# Autodesk Inventor assembly: RoboCinWheel
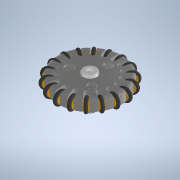
[picture p0: Inventor's stored thumbnail of the model, 180x180]
Saved by Autodesk Inventor 2020.4 (Build 244396000, 396)
## iProperties
Created: 2021-05-01
Part Number: RoboCinWheel
Document SubType Name: Assembly
Designer: Acer
Author: Acer
## Documents named in this file (10)
- C:\Users\Acer\Documents\MATLAB\Doutorado\CAD\Inventor\first_floor\Wheel\RoboCinWheel.iam
- C:\Users\Acer\Documents\MATLAB\Doutorado\CAD\Inventor\first_floor\Wheel\PartA.ipt
- C:\Users\Acer\Documents\MATLAB\Doutorado\CAD\Inventor\first_floor\Wheel\Wire.ipt
- C:\Users\Acer\Documents\MATLAB\Doutorado\CAD\Inventor\first_floor\Wheel\Roller.iam
- C:\Users\Acer\Documents\MATLAB\Doutorado\CAD\Inventor\first_floor\Wheel\gear_z60_26106000_machined.ipt
- C:\Users\Acer\Documents\MATLAB\Doutorado\CAD\Inventor\first_floor\Wheel\PartB.ipt
- C:\Users\Acer\Documents\MATLAB\Doutorado\CAD\Inventor\first_floor\Wheel\685-ZZ-C3.ipt
- C:\Users\Acer\Documents\MATLAB\Doutorado\CAD\Inventor\first_floor\Wheel\ScrewM5x40_Machined.ipt
- C:\Users\Acer\Documents\Inventor\Content Center Files\R2020\en-US\DIN 84\DIN 84 - M3 x 12.ipt
- C:\Users\Acer\Documents\Inventor\Content Center Files\R2020\en-US\DIN EN ISO 4032\DIN EN ISO 4032 - M3.ipt
## Components (33 placed, 9 different names)
1. PartA:1 — Rigid:1, Mate:1, Mate:2, Mate:3, Mate:4, Mate:5, Mate:6, Mate:7, Mate:8, Mate:24, Mate:25, Mate:26, Mate:27, Mate:28, Mate:29, Angle:4, Angle:5, Angle:6
2. Wire:1 — Rigid:1
3. gear_z60_26106000_machined:1 — Mate:2, Mate:3, Mate:4, Mate:9, Mate:12, Mate:13, Mate:14, Mate:15, Mate:16, Mate:17
4. PartB:1 — Mate:5, Mate:6, Mate:7, Mate:18, Mate:19, Mate:20, Mate:21, Mate:22, Mate:23, Angle:1, Angle:2, Angle:3
5. Kugellager 685-ZZ-C3:1 — Mate:8, Mate:9, Mate:10, Mate:11
6. ScrewM5x40_Machined:1 — Mate:10, Mate:11
7. DIN 84 - replaced by DIN EN ISO 1207 M3 x 12:1 — Mate:12, Mate:17
8. DIN 84 - replaced by DIN EN ISO 1207 M3 x 12:2 — Mate:13, Mate:15
9. DIN 84 - replaced by DIN EN ISO 1207 M3 x 12:3 — Mate:14, Mate:16
10. DIN EN ISO 4032 M3:1 — Mate:26, Mate:27, Angle:6
11. DIN EN ISO 4032 M3:2 — Mate:25, Mate:28, Angle:5
12. DIN EN ISO 4032 M3:3 — Mate:24, Mate:29, Angle:4
13. DIN EN ISO 4032 M3:4 — Mate:18, Mate:22, Angle:2
14. DIN EN ISO 4032 M3:5 — Mate:19, Mate:21, Angle:3
15. DIN EN ISO 4032 M3:6 — Mate:20, Mate:23, Angle:1
16. Roller:1 [sub-assembly] — Mate:1
17. Roller:2 [sub-assembly]
18. Roller:3 [sub-assembly]
19. Roller:4 [sub-assembly]
20. Roller:5 [sub-assembly]
21. Roller:6 [sub-assembly]
22. Roller:7 [sub-assembly]
23. Roller:8 [sub-assembly]
24. Roller:9 [sub-assembly]
25. Roller:10 [sub-assembly]
26. Roller:11 [sub-assembly]
27. Roller:12 [sub-assembly]
28. Roller:13 [sub-assembly]
29. Roller:14 [sub-assembly]
30. Roller:15 [sub-assembly]
31. Roller:16 [sub-assembly]
32. Roller:17 [sub-assembly]
33. Roller:18 [sub-assembly]
## Component patterns: (18 elements, first: Roller:1)
## Relationships (36: Mate 29, Angle 6, WeldJoint 1)
- Rigid:1 [WeldJoint] (1.2 mm): PartA:1 ↔ Wire:1
- Mate:1 (0.15 mm): PartA:1 ↔ Roller:1
- Mate:2: PartA:1 ↔ gear_z60_26106000_machined:1
- Mate:3: PartA:1 ↔ gear_z60_26106000_machined:1
- Mate:4: PartA:1 ↔ gear_z60_26106000_machined:1
- Mate:5: PartA:1 ↔ PartB:1
- Mate:6: PartA:1 ↔ PartB:1
- Mate:7: PartA:1 ↔ PartB:1
- Mate:8: PartA:1 ↔ Kugellager 685-ZZ-C3:1
- Mate:9: gear_z60_26106000_machined:1 ↔ Kugellager 685-ZZ-C3:1
- Mate:10: Kugellager 685-ZZ-C3:1 ↔ ScrewM5x40_Machined:1
- Mate:11: Kugellager 685-ZZ-C3:1 ↔ ScrewM5x40_Machined:1
- Mate:12: gear_z60_26106000_machined:1 ↔ DIN 84 - replaced by DIN EN ISO 1207 M3 x 12:1
- Mate:13: gear_z60_26106000_machined:1 ↔ DIN 84 - replaced by DIN EN ISO 1207 M3 x 12:2
- Mate:14: gear_z60_26106000_machined:1 ↔ DIN 84 - replaced by DIN EN ISO 1207 M3 x 12:3
- Mate:15: gear_z60_26106000_machined:1 ↔ DIN 84 - replaced by DIN EN ISO 1207 M3 x 12:2
- Mate:16: gear_z60_26106000_machined:1 ↔ DIN 84 - replaced by DIN EN ISO 1207 M3 x 12:3
- Mate:17: gear_z60_26106000_machined:1 ↔ DIN 84 - replaced by DIN EN ISO 1207 M3 x 12:1
- Mate:18: PartB:1 ↔ DIN EN ISO 4032 M3:4
- Mate:19: PartB:1 ↔ DIN EN ISO 4032 M3:5
- Mate:20: PartB:1 ↔ DIN EN ISO 4032 M3:6
- Mate:21: PartB:1 ↔ DIN EN ISO 4032 M3:5
- Mate:22: PartB:1 ↔ DIN EN ISO 4032 M3:4
- Mate:23: PartB:1 ↔ DIN EN ISO 4032 M3:6
- Angle:1 (0 deg): PartB:1 ↔ DIN EN ISO 4032 M3:6
- Angle:2 (0 deg): PartB:1 ↔ DIN EN ISO 4032 M3:4
- Angle:3 (0 deg): PartB:1 ↔ DIN EN ISO 4032 M3:5
- Mate:24: PartA:1 ↔ DIN EN ISO 4032 M3:3
- Mate:25: PartA:1 ↔ DIN EN ISO 4032 M3:2
- Mate:26: PartA:1 ↔ DIN EN ISO 4032 M3:1
- Mate:27: PartA:1 ↔ DIN EN ISO 4032 M3:1
- Mate:28: PartA:1 ↔ DIN EN ISO 4032 M3:2
- Mate:29: PartA:1 ↔ DIN EN ISO 4032 M3:3
- Angle:4 (0 deg): PartA:1 ↔ DIN EN ISO 4032 M3:3
- Angle:5 (0 deg): PartA:1 ↔ DIN EN ISO 4032 M3:2
- Angle:6 (0 deg): PartA:1 ↔ DIN EN ISO 4032 M3:1
